# Autodesk Inventor assembly: sorterbucket
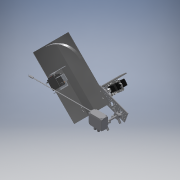
[picture p0: Inventor's stored thumbnail of the model, 180x180]
Saved by Autodesk Inventor 2019 (Build 230136000, 136)
## iProperties
Created: 2018-12-06
Part Number: sorterbucket
Document SubType Name: Assembly
Designer: User
Mass: 469.407 g
Surface Area: 1803.04 cm^2
Volume: 197.417 cm^3
Density: 2.37774 g/cm^3
Author: User
## Documents named in this file (11)
- C:\Robotics\CAD\2018-19_CAD\Collection\sorterbucket vex servo.iam
- C:\Robotics\CAD\2018-19_CAD\Collection\Sorter.ipt
- C:\Robotics\CAD\COTSParts\Actobotics\585 parts\585580FlatTriplePatternBracket.ipt
- C:\Robotics\CAD\COTSParts\Tetrix\39274_txm-flat64mmx27mm.ipt
- C:\Robotics\CAD\COTSParts\Tetrix\Tetrix servo 180.ipt
- C:\Robotics\CAD\COTSParts\Tetrix\39060_txm-standard servo bracket.ipt
- C:\Robotics\CAD\COTSParts\Actobotics\634 parts\634078.25inDShaft3.5inLong.ipt
- C:\Robotics\CAD\2018-19_CAD\Collection\SweeperHub.ipt
- C:\Robotics\CAD\2018-19_CAD\smart servo with servo block.iam
- C:\Robotics\CAD\2018-19_CAD\Collection\bucket holder plate.ipt
- C:\Robotics\CAD\COTSParts\Vex\2-Wire_Motor_393_276-2177.iam
## Components (11 placed, 10 different names)
1. Sorter:1 — Mate:1, Mate:27, Mate:28, Flush:4, Mate:40, Mate:41, Angle:5
2. 585580FlatTriplePatternBracket:1 — Mate:1, Mate:13, Mate:23, Mate:24, Angle:5, Mate:43
3. 634078.25inDShaft3.5inLong:1 — Mate:13, Mate:21, Mate:22, Angle:4, Mate:40, Mate:41
4. SweeperHub:1 — Mate:22, Flush:2
5. SweeperHub:2 — Mate:21, Flush:2, Angle:4, Mate:43
6. smart servo with servo block:1 [sub-assembly] — Mate:23, Mate:24, Mate:42, Flush:9, Flush:10
7. Tetrix servo 180:1 — Mate:27, Mate:29, Mate:30, Angle:3, Mate:33, Mate:34
8. 39060_txm-standard servo bracket:2 — Mate:28, Mate:29, Mate:30, Angle:3, Flush:4
9. 39274_txm-flat64mmx27mm:2 — Mate:33, Mate:34
10. bucket holder plate:1 — Mate:42, Flush:9, Flush:10
11. 2-Wire_Motor_393_276-2177:1 [sub-assembly]
## Relationships (23: Mate 16, Flush 4, Angle 3)
- Mate:1: Sorter:1 ↔ 585580FlatTriplePatternBracket:1
- Mate:13: 585580FlatTriplePatternBracket:1 ↔ 634078.25inDShaft3.5inLong:1
- Mate:21: 634078.25inDShaft3.5inLong:1 ↔ SweeperHub:2
- Mate:22: 634078.25inDShaft3.5inLong:1 ↔ SweeperHub:1
- Flush:2: SweeperHub:1 ↔ SweeperHub:2
- Mate:23: 585580FlatTriplePatternBracket:1 ↔ smart servo with servo block:1
- Mate:24: 585580FlatTriplePatternBracket:1 ↔ smart servo with servo block:1
- Mate:27: Sorter:1 ↔ Tetrix servo 180:1
- Mate:28: Sorter:1 ↔ 39060_txm-standard servo bracket:2
- Mate:29: Tetrix servo 180:1 ↔ 39060_txm-standard servo bracket:2
- Mate:30: Tetrix servo 180:1 ↔ 39060_txm-standard servo bracket:2
- Angle:3 (0 deg): Tetrix servo 180:1 ↔ 39060_txm-standard servo bracket:2
- Flush:4: Sorter:1 ↔ 39060_txm-standard servo bracket:2
- Mate:33: Tetrix servo 180:1 ↔ 39274_txm-flat64mmx27mm:2
- Mate:34: Tetrix servo 180:1 ↔ 39274_txm-flat64mmx27mm:2
- Angle:4 (0 deg): 634078.25inDShaft3.5inLong:1 ↔ SweeperHub:2
- Mate:40 (97.79 mm): Sorter:1 ↔ 634078.25inDShaft3.5inLong:1
- Mate:41 (38.1 mm): Sorter:1 ↔ 634078.25inDShaft3.5inLong:1
- Angle:5 (-25 deg): Sorter:1 ↔ 585580FlatTriplePatternBracket:1
- Mate:42: smart servo with servo block:1 ↔ bucket holder plate:1
- Flush:9: smart servo with servo block:1 ↔ bucket holder plate:1
- Flush:10: smart servo with servo block:1 ↔ bucket holder plate:1
- Mate:43 (12.7 mm): 585580FlatTriplePatternBracket:1 ↔ SweeperHub:2
